# Autodesk Inventor assembly: 300-031 (BODY SUPPORT)
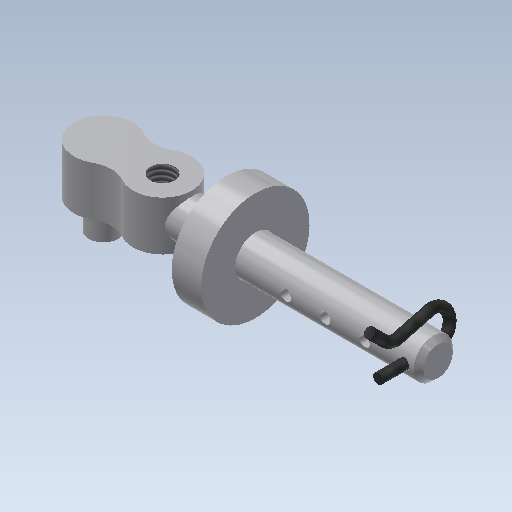
[picture p0: Inventor's stored thumbnail of the model, 512x512]
Saved by Autodesk Inventor 2020 (Build 240168000, 168)
## iProperties
Created: 2015-04-18
Part Number: 300-031 (BODY SUPPORT)
Document SubType Name: Assembly
Designer: Station9
Author: Station9
## Documents named in this file (4)
- C:\Users\0x6f736f646f\Downloads\rc-car-16.snapshot.3\300-031 (BODY SUPPORT).iam
- C:\Users\0x6f736f646f\Downloads\rc-car-16.snapshot.3\500-178.ipt
- C:\Users\0x6f736f646f\Downloads\rc-car-16.snapshot.3\500-177.ipt
- C:\Users\0x6f736f646f\Downloads\rc-car-16.snapshot.3\500-179.ipt
## Components (3 placed, 3 different names)
1. 500-178:1 — Mate:1, Mate:2
2. 500-177:1 — Mate:2
3. 500-179:1 — Mate:1
## Relationships (2: Mate 2)
- Mate:1: 500-178:1 ↔ 500-179:1
- Mate:2: 500-178:1 ↔ 500-177:1
